# Autodesk Inventor assembly: ASY LASER
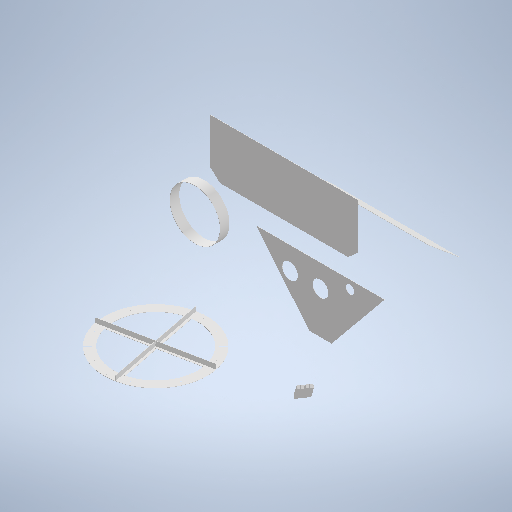
[picture p0: Inventor's stored thumbnail of the model, 512x512]
Saved by Autodesk Inventor 2025 (Build 290162010, 162A)
## iProperties
Created: 2024-09-04
Part Number: ASY LASER
Document SubType Name: Assembly
Designer: admin
Author: admin
## Documents named in this file (7)
- C:\Users\DELL\YandexDisk-badmisterfox\домашниий пк\Inventor\Manturovo\Manturovo_Se-clar\DXF файлы\ASY LASER.iam
- C:\Users\DELL\YandexDisk-badmisterfox\домашниий пк\Inventor\Manturovo\Manturovo_Se-clar\MSC 402 ring.ipt
- C:\Users\DELL\YandexDisk-badmisterfox\домашниий пк\Inventor\Manturovo\АРХИВНЫЙ Manturovo_Se-clar\конус\MSC 074 face 1.ipt
- C:\Users\DELL\YandexDisk-badmisterfox\домашниий пк\Inventor\Manturovo\АРХИВНЫЙ Manturovo_Se-clar\MSC 075 face 2.ipt
- C:\Users\DELL\YandexDisk-badmisterfox\домашниий пк\Inventor\Manturovo\АРХИВНЫЙ Manturovo_Se-clar\MSC 076 face 3.ipt
- C:\Users\DELL\YandexDisk-badmisterfox\домашниий пк\Inventor\Manturovo\Manturovo_Se-clar\DXF файлы\Workspaces\Workspace\ASY BSH 500 cap.iam
- C:\Users\DELL\YandexDisk-badmisterfox\домашниий пк\Inventor\Manturovo\АРХИВНЫЙ Manturovo_Se-clar\MSC 128 flange base tube support_CPY.ipt
## Components (13 placed, 6 different names)
1. MSC 402 ring:1
2. MSC 074 face 1:1
3. MSC 075 face 2:1
4. MSC 076 face 3:1
5. ASY BSH 500 cap:1 [sub-assembly]
6. MSC 128 flange base tube support_CPY:1
7. MSC 128 flange base tube support_CPY:2
8. MSC 128 flange base tube support_CPY:3
9. MSC 128 flange base tube support_CPY:4
10. MSC 128 flange base tube support_CPY:5
11. MSC 128 flange base tube support_CPY:6
12. MSC 128 flange base tube support_CPY:7
13. MSC 128 flange base tube support_CPY:8
## Component patterns: (8 elements, first: MSC 128 flange base tube support_CPY:1)
